# Autodesk Inventor assembly: Code Ring
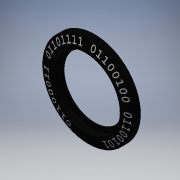
[picture p0: Inventor's stored thumbnail of the model, 180x180]
Saved by Autodesk Inventor 2016 (Build 200138000, 138)
## iProperties
Created: 2015-06-02
Part Number: Code Ring
Document SubType Name: Assembly
Designer: Spooner
Author: Spooner
## Documents named in this file (3)
- C:\Users\Spooner\Documents\Inventor\2016 RoboCat\Code Ring.iam
- C:\Users\Spooner\Documents\Inventor\2016 RoboCat\Team Pin Code.ipt
- C:\Users\Spooner\Documents\Inventor\2016 RoboCat\Team Pin Code-numbers.ipt
## Components (2 placed, 2 different names)
1. Team Pin Code:1 — Mate:10, Mate:11, Mate:12
2. Team Pin Code-numbers:1 — Mate:10, Mate:11, Mate:12
## Relationships (3: Mate 3)
- Mate:10: Team Pin Code:1 ↔ Team Pin Code-numbers:1
- Mate:11: Team Pin Code:1 ↔ Team Pin Code-numbers:1
- Mate:12: Team Pin Code:1 ↔ Team Pin Code-numbers:1
